# Autodesk Inventor assembly: Kitai
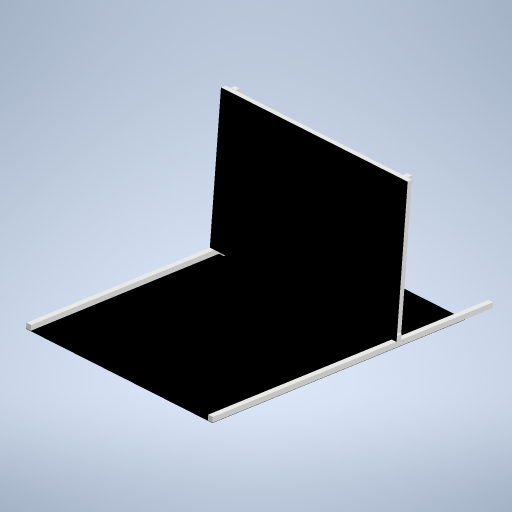
[picture p0: Inventor's stored thumbnail of the model, 512x512]
Saved by Autodesk Inventor 2023 (Build 270158000, 158)
## iProperties
Created: 2022-10-15
Part Number: Kitai
Document SubType Name: Assembly
Designer: banru
Author: banru
## Documents named in this file (6)
- C:\Users\banru\Documents\workspace\Contactless\Inventor\Kitai.iam
- C:\Users\banru\Documents\workspace\Contactless\Inventor\Dai.ipt
- C:\Users\banru\Documents\workspace\Contactless\Inventor\Yoko.ipt
- C:\Users\banru\Documents\workspace\Contactless\Inventor\Tate.ipt
- C:\Users\banru\Documents\workspace\Contactless\Inventor\Ita.ipt
- C:\Users\banru\Documents\workspace\Contactless\Inventor\YokoUe.ipt
## Components (9 placed, 5 different names)
1. Dai:1 — 挿入:2, 挿入:3
2. Dai:2 — メイト:7, メイト:8, フラッシュ:16, 挿入:1, 挿入:8, メイト:11, フラッシュ:17
3. Yoko:1 — 挿入:1, 挿入:2, メイト:10
4. Tate:1 — 挿入:3, 挿入:10
5. Ita:1 — メイト:12, フラッシュ:18, フラッシュ:19
6. Ita:2 — メイト:7, メイト:9, メイト:11, フラッシュ:17
7. Ita:4 — メイト:8, メイト:9, フラッシュ:16
8. YokoUe:1 — 挿入:9, 挿入:10, メイト:12, フラッシュ:18, フラッシュ:19
9. Tate:2 — 挿入:8, メイト:10, 挿入:9
## Relationships (16: Mate 6, Insert 6, Flush 4)
- メイト:7 [Mate]: Dai:2 ↔ Ita:2
- メイト:8 [Mate]: Dai:2 ↔ Ita:4
- メイト:9 [Mate]: Ita:2 ↔ Ita:4
- フラッシュ:16 [Flush]: Dai:2 ↔ Ita:4
- 挿入:1 [Insert]: Dai:2 ↔ Yoko:1
- 挿入:2 [Insert]: Dai:1 ↔ Yoko:1
- 挿入:3 [Insert]: Dai:1 ↔ Tate:1
- 挿入:8 [Insert]: Dai:2 ↔ Tate:2
- メイト:10 [Mate]: Yoko:1 ↔ Tate:2
- 挿入:9 [Insert]: YokoUe:1 ↔ Tate:2
- 挿入:10 [Insert]: Tate:1 ↔ YokoUe:1
- メイト:11 [Mate]: Dai:2 ↔ Ita:2
- フラッシュ:17 [Flush]: Dai:2 ↔ Ita:2
- メイト:12 [Mate]: Ita:1 ↔ YokoUe:1
- フラッシュ:18 [Flush]: Ita:1 ↔ YokoUe:1
- フラッシュ:19 [Flush]: Ita:1 ↔ YokoUe:1
